# Autodesk Inventor assembly: Assembly1
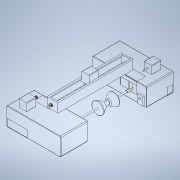
[picture p0: Inventor's stored thumbnail of the model, 180x180]
Saved by Autodesk Inventor 2020 (Build 240168000, 168)
## iProperties
Created: 2022-12-14
Part Number: Assembly1
Document SubType Name: Assembly
Designer: Manish
Author: Manish
## Documents named in this file (17)
- D:\my stuff\TYProject\cad\Assembly1.iam
- D:\my stuff\TYProject\cad\wheel.ipt
- D:\my stuff\TYProject\cad\WheelShaft.ipt
- D:\my stuff\TYProject\cad\batt.ipt
- D:\my stuff\TYProject\cad\motor.ipt
- D:\my stuff\TYProject\cad\motorCoupling5_8.ipt
- D:\my stuff\TYProject\cad\motor_MIR.ipt
- D:\my stuff\TYProject\cad\motorCoupling5_8_MIR.ipt
- D:\my stuff\TYProject\cad\stepper driver.ipt
- D:\my stuff\TYProject\cad\esp32CAM.ipt
- D:\my stuff\TYProject\cad\esp32CAM_MIR.ipt
- D:\my stuff\TYProject\cad\body.ipt
- D:\my stuff\TYProject\cad\motormount.ipt
- D:\my stuff\TYProject\cad\balancingFrame.ipt
- D:\my stuff\TYProject\cad\mass.ipt
- D:\my stuff\TYProject\cad\balanceRod.ipt
- D:\my stuff\TYProject\cad\pulley20.ipt
## Components (25 placed, 16 different names)
1. wheel:1 — Mate:1, Flush:1, Mate:2, Mate:3, Flush:25
2. wheel:2 — Mate:1, Flush:1, Mate:4, Mate:5
3. WheelShaft:1 — Mate:2, Mate:3, Flush:3, Mate:10, Mate:18, Symmetry:1, Mate:21, Flush:25, Flush:37
4. WheelShaft:2 — Mate:4, Mate:5, Mate:14, Mate:15, Mate:18, Symmetry:1, Mate:20
5. batt:1 — Flush:21, Flush:22, Flush:23
6. motor:2 — Flush:4, Mate:16, Flush:8, Flush:15, Flush:27, Mate:24, Flush:29, Flush:30
7. motorCoupling5_8:2 — Flush:3, Mate:10
8. motor_MIR:1 — Mate:12, Mate:13, Flush:4, Mate:17, Flush:10, Flush:16, Flush:26, Flush:28, Flush:31, Flush:32
9. motorCoupling5_8_MIR:1 — Mate:12, Mate:13, Mate:14, Mate:15
10. batt:2 — Flush:19, Flush:20, Flush:24
11. stepper driver:1 — Mate:16, Flush:8, Flush:27
12. stepper driver:2 — Mate:17, Flush:10, Flush:26
13. esp32CAM:1 — Flush:35, Mate:25, Flush:38
14. esp32CAM_MIR:1 — Mate:22, Flush:36, Flush:38
15. body:1 — Flush:14, Flush:15, Symmetry:2, Mate:20, Flush:21, Flush:22, Flush:23, Flush:34, Flush:35, Mate:26, Symmetry:3, Mate:32
16. body:2 — Flush:14, Flush:16, Symmetry:2, Mate:21, Flush:19, Flush:20, Flush:24, Mate:22, Flush:33, Flush:36, Symmetry:3, Mate:35
17. motormount:1 — Flush:28, Flush:31, Flush:32, Flush:33
18. motormount:2 — Mate:24, Flush:29, Flush:30, Flush:34
19. balancingFrame:1 — Mate:26, Mate:27, Mate:28, Mate:29, Mate:30, Mate:37
20. mass:1 — Mate:29, Mate:30, Flush:39, Mate:31
21. balanceRod:1 — Mate:31, Flush:40, Mate:34, Mate:37, Mate:38
22. pulley20:1 — Flush:40, Flush:42, Mate:34, Mate:38
23. motor:3 — Mate:32, Flush:41, Mate:33, Symmetry:4, Symmetry:5
24. pulley20:2 — Flush:41, Mate:33, Flush:42
25. motor:4 — Mate:35, Symmetry:4, Symmetry:5
## Relationships (70: Mate 33, Flush 32, Symmetry 5)
- Mate:1: wheel:1 ↔ wheel:2
- Flush:1: wheel:1 ↔ wheel:2
- Mate:2: wheel:1 ↔ WheelShaft:1
- Mate:3: wheel:1 ↔ WheelShaft:1
- Mate:4: wheel:2 ↔ WheelShaft:2
- Mate:5: wheel:2 ↔ WheelShaft:2
- [Mate]: motor:2 ↔ motorCoupling5_8:2
- [Mate]: motor:2 ↔ motorCoupling5_8:2
- Flush:3: WheelShaft:1 ↔ motorCoupling5_8:2
- Mate:10: WheelShaft:1 ↔ motorCoupling5_8:2
- Mate:12: motor_MIR:1 ↔ motorCoupling5_8_MIR:1
- Mate:13: motor_MIR:1 ↔ motorCoupling5_8_MIR:1
- Mate:14: WheelShaft:2 ↔ motorCoupling5_8_MIR:1
- Mate:15: WheelShaft:2 ↔ motorCoupling5_8_MIR:1
- Flush:4: motor:2 ↔ motor_MIR:1
- Mate:16: motor:2 ↔ stepper driver:1
- Flush:8: motor:2 ↔ stepper driver:1
- Mate:17: motor_MIR:1 ↔ stepper driver:2
- Flush:10: motor_MIR:1 ↔ stepper driver:2
- Mate:18 (-150 mm): WheelShaft:1 ↔ WheelShaft:2
- Flush:14: body:1 ↔ body:2
- Flush:15: motor:2 ↔ body:1
- Flush:16: motor_MIR:1 ↔ body:2
- Symmetry:1: WheelShaft:1 ↔ WheelShaft:2
- Symmetry:2: body:1 ↔ body:2
- Mate:19
- Mate:20: WheelShaft:2 ↔ body:1
- Mate:21: WheelShaft:1 ↔ body:2
- Flush:19: batt:2 ↔ body:2
- Flush:20: batt:2 ↔ body:2
- Flush:21: batt:1 ↔ body:1
- Flush:22: batt:1 ↔ body:1
- Flush:23: batt:1 ↔ body:1
- Flush:24: batt:2 ↔ body:2
- Mate:22: esp32CAM_MIR:1 ↔ body:2
- Flush:25: wheel:1 ↔ WheelShaft:1
- Flush:26: motor_MIR:1 ↔ stepper driver:2
- Flush:27: motor:2 ↔ stepper driver:1
- Flush:28: motor_MIR:1 ↔ motormount:1
- Mate:24: motor:2 ↔ motormount:2
- Flush:29: motor:2 ↔ motormount:2
- Flush:30: motor:2 ↔ motormount:2
- Flush:31: motor_MIR:1 ↔ motormount:1
- Flush:32: motor_MIR:1 ↔ motormount:1
- Flush:33: body:2 ↔ motormount:1
- Flush:34: body:1 ↔ motormount:2
- Flush:35 (10 mm): esp32CAM:1 ↔ body:1
- Flush:36 (-10 mm): esp32CAM_MIR:1 ↔ body:2
- Flush:37 (20 mm): WheelShaft:1
- Mate:25: esp32CAM:1
- Flush:38: esp32CAM:1 ↔ esp32CAM_MIR:1
- Mate:26: body:1 ↔ balancingFrame:1
- Symmetry:3: body:1 ↔ body:2
- Mate:27: balancingFrame:1
- Mate:28: balancingFrame:1
- Mate:29: balancingFrame:1 ↔ mass:1
- Mate:30: balancingFrame:1 ↔ mass:1
- Flush:39: mass:1
- Mate:31: mass:1 ↔ balanceRod:1
- Flush:40: balanceRod:1 ↔ pulley20:1
- Mate:32: body:1 ↔ motor:3
- Flush:41: motor:3 ↔ pulley20:2
- Mate:33: motor:3 ↔ pulley20:2
- Flush:42: pulley20:1 ↔ pulley20:2
- Mate:34: balanceRod:1 ↔ pulley20:1
- Mate:35: body:2 ↔ motor:4
- Symmetry:4: motor:3 ↔ motor:4
- Mate:37: balancingFrame:1 ↔ balanceRod:1
- Symmetry:5: motor:3 ↔ motor:4
- Mate:38: balanceRod:1 ↔ pulley20:1
## Named parameters: d16_d14 = 0 mm, d17_d15 = 0 mm
